# Autodesk Inventor assembly: A
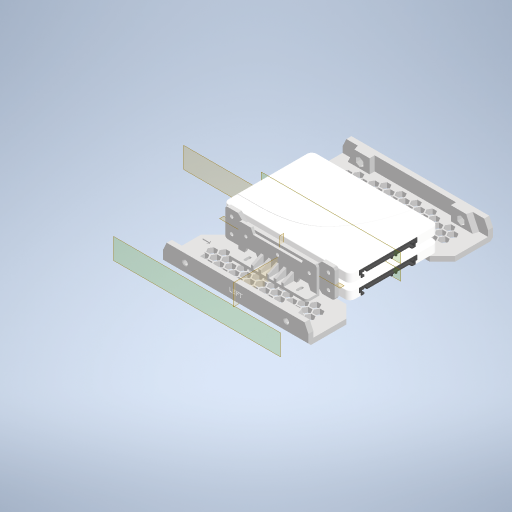
[picture p0: Inventor's stored thumbnail of the model, 512x512]
Saved by Autodesk Inventor 2023 (Build 270158000, 158)
## iProperties
Created: 2022-06-11
Part Number: A
Document SubType Name: Assembly
Designer: kfcs7
Author: kfcs7
## Documents named in this file (6)
- E:\Github\5.25-Bay-Adapter\A.iam
- E:\Github\5.25-Bay-Adapter\A-02.ipt
- E:\Github\5.25-Bay-Adapter\A-03.ipt
- E:\Github\5.25-Bay-Adapter\A-04.ipt
- E:\Github\5.25-Bay-Adapter\A-06.ipt
- E:\Github\5.25-Bay-Adapter\A-07.ipt
## Components (6 placed, 5 different names)
1. A-02:1 — Rigid:1, Symmetry:1
2. A-03:1 — Rigid:1, Symmetry:1, Flush:4, Mate:2
3. A-06:1 — Flush:3, Flush:4, Mate:2, Flush:5
4. A-07:1 — Flush:5
5. A-04:1 — Flush:2, Mate:1
6. A-04:2 — Flush:3
## Component patterns: (2 elements, first: A-04:1)
## Relationships (8: Flush 4, Mate 2, WeldJoint 1, Symmetry 1)
- Rigid:1 [WeldJoint] (-146 mm): A-02:1 ↔ A-03:1
- Flush:2: A-04:1
- Flush:3: A-06:1 ↔ A-04:2
- Symmetry:1: A-02:1 ↔ A-03:1
- Mate:1: A-04:1
- Flush:4: A-03:1 ↔ A-06:1
- Mate:2 (2.5 mm): A-03:1 ↔ A-06:1
- Flush:5: A-06:1 ↔ A-07:1
